# Autodesk Inventor assembly: zespol_z_lozyskami
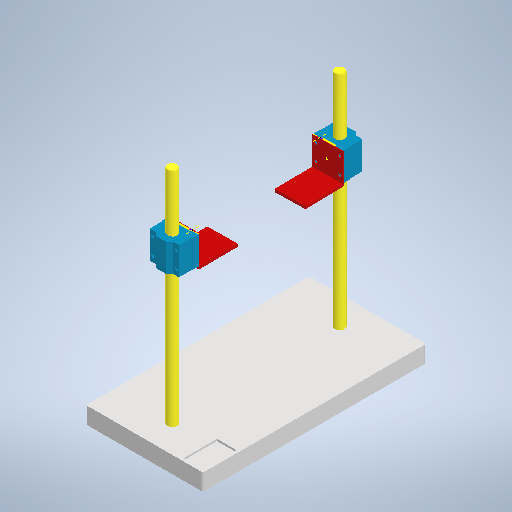
[picture p0: Inventor's stored thumbnail of the model, 512x512]
Saved by Autodesk Inventor 2025 (Build 290162000, 162)
## iProperties
Created: 2024-04-05
Part Number: zespol_z_lozyskami
Document SubType Name: Assembly
Designer: Wojtek
Author: Wojtek
## Documents named in this file (5)
- C:\Users\Wojtek\Documents\zespol_z_lozyskami.iam
- C:\Users\Wojtek\Documents\Podstawa.ipt
- C:\Users\Wojtek\Documents\pret_pionowy.ipt
- C:\Users\Wojtek\Documents\lozysko.ipt
- C:\Users\Wojtek\Downloads\obudowa_łoż_pion_1.ipt
## Components (7 placed, 4 different names)
1. Podstawa:1 — Insert:1, Insert:2
2. pret_pionowy:1 — Insert:2, Insert:4
3. pret_pionowy:2 — Insert:1, Insert:3, Flush:1
4. lozysko:1 — Insert:3, Flush:1, Insert:5, Insert:9
5. lozysko:2 — Insert:4, Insert:7, Insert:8
6. obudowa_łoż_pion_1:1 — Insert:7, Insert:8
7. obudowa_łoż_pion_1:2 — Insert:5, Insert:9
## Relationships (9: Insert 8, Flush 1)
- Insert:1: Podstawa:1 ↔ pret_pionowy:2
- Insert:2: Podstawa:1 ↔ pret_pionowy:1
- Insert:3 (100 mm): pret_pionowy:2 ↔ lozysko:1
- Insert:4 (100 mm): pret_pionowy:1 ↔ lozysko:2
- Flush:1: pret_pionowy:2 ↔ lozysko:1
- Insert:5 (-2 mm): lozysko:1 ↔ obudowa_łoż_pion_1:2
- Insert:7 (-2 mm): lozysko:2 ↔ obudowa_łoż_pion_1:1
- Insert:8 (-2 mm): lozysko:2 ↔ obudowa_łoż_pion_1:1
- Insert:9 (-2 mm): lozysko:1 ↔ obudowa_łoż_pion_1:2
